# Autodesk Inventor assembly: Ball
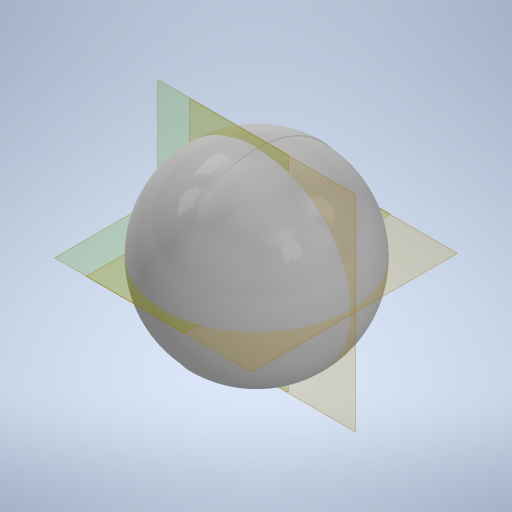
[picture p0: Inventor's stored thumbnail of the model, 512x512]
Saved by Autodesk Inventor 2024 (Build 280153000, 153)
## iProperties
Created: 2023-06-14
Part Number: Ball
Document SubType Name: Assembly
Designer: kakik
Author: kakik
## Documents named in this file (3)
- C:\Users\kakik\OneDrive\Desktop\p2\Ball\Ball.iam
- C:\Users\kakik\OneDrive\Desktop\p2\Ball\sphere-hollow-sphere1-thread-inner.ipt
- C:\Users\kakik\OneDrive\Desktop\p2\Ball\sphere-hollow-sphere1-thread-outer.ipt
## Components (2 placed, 2 different names)
1. sphere-hollow-sphere1-thread-inner:1 — Mate:1, Mate:2, Mate:3
2. sphere-hollow-sphere1-thread-outer:1 — Mate:1, Mate:2, Mate:3
## Relationships (3: Mate 3)
- Mate:1: sphere-hollow-sphere1-thread-inner:1 ↔ sphere-hollow-sphere1-thread-outer:1
- Mate:2: sphere-hollow-sphere1-thread-inner:1 ↔ sphere-hollow-sphere1-thread-outer:1
- Mate:3: sphere-hollow-sphere1-thread-inner:1 ↔ sphere-hollow-sphere1-thread-outer:1
